# Autodesk Inventor assembly: Base (Draft 2)
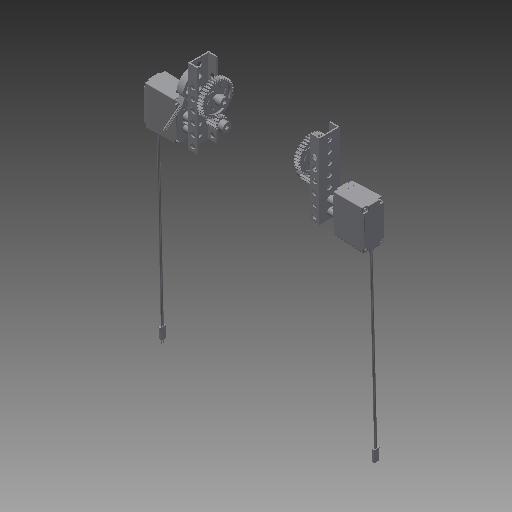
[picture p0: Inventor's stored thumbnail of the model, 512x512]
Saved by Autodesk Inventor 2018 (Build 220112000, 112)
## iProperties
Created: 2017-06-28
Part Number: Base (Draft 2)
Document SubType Name: Assembly
Designer: James
Author: James
## Documents named in this file (7)
- C:\Users\James\Desktop\EE REU\Hardware\Vex Arm\Vex Arm Draft 2\Base (Draft 2).iam
- C:\Users\James\Desktop\EE REU\Hardware\Vex Arm\Vex Parts\Base C Channel.ipt
- C:\Users\James\Desktop\EE REU\Hardware\Vex Arm\Vex Parts\393motor.ipt
- C:\Users\James\Desktop\EE REU\Hardware\Vex Arm\Vex Parts\Vex Gear Kit\VEX-36-TOOTH-GEAR.ipt
- C:\Users\James\Desktop\EE REU\Hardware\Vex Arm\Vex Parts\12 Tooth Metal Pinion.ipt
- C:\Users\James\Desktop\EE REU\Hardware\Vex Arm\Vex Parts\MOTION-MODEL-PACK\SHAFT-COLLAR.ipt
- C:\Users\James\Desktop\EE REU\Hardware\Vex Arm\Vex Parts\Vex Potentiometer.ipt
## Components (15 placed, 6 different names)
1. Base C Channel:1 — Flush:1, Flush:2, Insert:2, Insert:3, Insert:4, Insert:11, Mate:1
2. Base C Channel:2 — Flush:1, Flush:2, Insert:1, Insert:6, Insert:7, Mate:1
3. 393motor:1 — Insert:2
4. 393motor:2 — Insert:1
5. VEX-36-TOOTH-GEAR:1 — Insert:7, Insert:8, Insert:10
6. VEX-36-TOOTH-GEAR:2 — Insert:4, Insert:5, Insert:9
7. 12 Tooth Metal Pinion:1 — Insert:3, Insert:12
8. 12 Tooth Metal Pinion:2 — Insert:6, Insert:13
9. SHAFT-COLLAR:1 — Insert:10
10. SHAFT-COLLAR:2 — Insert:9
11. SHAFT-COLLAR:3 — Insert:13
12. SHAFT-COLLAR:4 — Insert:5
13. SHAFT-COLLAR:5 — Insert:8
14. SHAFT-COLLAR:6 — Insert:12
15. Vex Potentiometer:1 — Insert:11
## Relationships (16: Insert 13, Flush 2, Mate 1)
- Flush:1: Base C Channel:1 ↔ Base C Channel:2
- Flush:2: Base C Channel:1 ↔ Base C Channel:2
- Insert:1: Base C Channel:2 ↔ 393motor:2
- Insert:2: Base C Channel:1 ↔ 393motor:1
- Insert:3 (15 mm): Base C Channel:1 ↔ 12 Tooth Metal Pinion:1
- Insert:4 (15 mm): Base C Channel:1 ↔ VEX-36-TOOTH-GEAR:2
- Insert:5: VEX-36-TOOTH-GEAR:2 ↔ SHAFT-COLLAR:4
- Insert:6 (15 mm): Base C Channel:2 ↔ 12 Tooth Metal Pinion:2
- Insert:7 (15 mm): Base C Channel:2 ↔ VEX-36-TOOTH-GEAR:1
- Insert:8: VEX-36-TOOTH-GEAR:1 ↔ SHAFT-COLLAR:5
- Insert:9: VEX-36-TOOTH-GEAR:2 ↔ SHAFT-COLLAR:2
- Insert:10: VEX-36-TOOTH-GEAR:1 ↔ SHAFT-COLLAR:1
- Insert:11: Base C Channel:1 ↔ Vex Potentiometer:1
- Insert:12: 12 Tooth Metal Pinion:1 ↔ SHAFT-COLLAR:6
- Insert:13: 12 Tooth Metal Pinion:2 ↔ SHAFT-COLLAR:3
- Mate:1 (160 mm): Base C Channel:1 ↔ Base C Channel:2
